# Autodesk Inventor assembly: clip
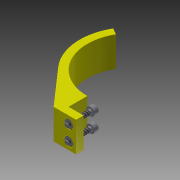
[picture p0: Inventor's stored thumbnail of the model, 180x180]
Saved by Autodesk Inventor 2013 (Build 170138000, 138)
## iProperties
Created: 2013-12-08
Part Number: clip
Document SubType Name: Assembly
Designer: employee
Author: employee
## Documents named in this file (4)
- C:\Users\employee\Desktop\linear simpson 3\clip.iam
- C:\Users\employee\Desktop\linear simpson 3\clip.ipt
- C:\Users\employee\Desktop\linear simpson 3\M3 NUT.ipt
- C:\Users\employee\Desktop\linear simpson 3\M3x16.ipt
## Components (5 placed, 3 different names)
1. clip:1 — Insert:1, Insert:2, Insert:3, Insert:4, Angle:1, Angle:2
2. M3 NUT:1 — Insert:3, Angle:1
3. M3 NUT:2 — Insert:4, Angle:2
4. M3x16:1 — Insert:1
5. M3x16:2 — Insert:2
## Relationships (6: Insert 4, Angle 2)
- Insert:1 (9.5 mm): clip:1 ↔ M3x16:1
- Insert:2 (9.5 mm): clip:1 ↔ M3x16:2
- Insert:3: clip:1 ↔ M3 NUT:1
- Insert:4: clip:1 ↔ M3 NUT:2
- Angle:1 (0 deg): clip:1 ↔ M3 NUT:1
- Angle:2 (0 deg): clip:1 ↔ M3 NUT:2
